# Autodesk Inventor assembly: Plate Assembly
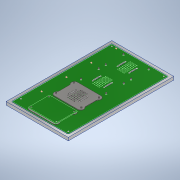
[picture p0: Inventor's stored thumbnail of the model, 180x180]
Saved by Autodesk Inventor 2022 (Build 260153000, 153)
## iProperties
Created: 2021-07-29
Part Number: Plate Assembly
Document SubType Name: Assembly
Designer: Caleb
Author: Caleb
## Documents named in this file (7)
- C:\Users\Caleb\Desktop\nebraska-silicon-lab\Hardware\ETL\Module Assembly\Tamale Assembly Plate V2\Plate Assembly.iam
- C:\Users\Caleb\Desktop\nebraska-silicon-lab\Hardware\ETL\Module Assembly\Tamale Assembly Plate V2\Tamale Assembly Plate.ipt
- C:\Users\Caleb\Desktop\nebraska-silicon-lab\Hardware\ETL\Module Assembly\Tamale Assembly Plate V2\91585A353_18-8 STAINLESS STEEL DOWEL PIN.ipt
- C:\Users\Caleb\Desktop\nebraska-silicon-lab\Hardware\ETL\Module Assembly\Tamale Assembly Plate V2\90910A443_BUTTON HEAD TORX SCREWS.ipt
- C:\Users\Caleb\Desktop\nebraska-silicon-lab\Hardware\ETL\Module Assembly\Tamale Assembly Plate V2\spacer.ipt
- C:\Users\Caleb\Desktop\nebraska-silicon-lab\Hardware\ETL\Module Assembly\Module PCB Mockup\etl_module_pcb_mockup_v1.iam
- C:\Users\Caleb\Desktop\nebraska-silicon-lab\Hardware\ETL\Module Assembly\Tamale Assembly Plate V2\etl_assembly_plate_pcb_v1.1\etl_assembly_plate_pcb_v1.iam
## Components (41 placed, 6 different names)
1. Tamale Assembly Plate:1 — Insert:1, Insert:2, Insert:3, Insert:4, Insert:5, Insert:6, Insert:7, Insert:8, Insert:9, Insert:10, Insert:11, Insert:12, Insert:13, Insert:14, Insert:15, Insert:16, Mate:5, Insert:17, Insert:18
2. 91585A353_18-8 STAINLESS STEEL DOWEL PIN:1 — Insert:2
3. 91585A353_18-8 STAINLESS STEEL DOWEL PIN:2 — Insert:3
4. 91585A353_18-8 STAINLESS STEEL DOWEL PIN:3 — Insert:4
5. 91585A353_18-8 STAINLESS STEEL DOWEL PIN:4 — Insert:1
6. 91585A353_18-8 STAINLESS STEEL DOWEL PIN:5 — Insert:8
7. 91585A353_18-8 STAINLESS STEEL DOWEL PIN:6 — Insert:7
8. 91585A353_18-8 STAINLESS STEEL DOWEL PIN:7 — Insert:6
9. 91585A353_18-8 STAINLESS STEEL DOWEL PIN:8 — Insert:5
10. 91585A353_18-8 STAINLESS STEEL DOWEL PIN:9 — Insert:9
11. 91585A353_18-8 STAINLESS STEEL DOWEL PIN:11 — Insert:10
12. 91585A353_18-8 STAINLESS STEEL DOWEL PIN:12 — Insert:16
13. 91585A353_18-8 STAINLESS STEEL DOWEL PIN:13 — Insert:15
14. 91585A353_18-8 STAINLESS STEEL DOWEL PIN:14 — Insert:13
15. 91585A353_18-8 STAINLESS STEEL DOWEL PIN:15 — Insert:12
16. 91585A353_18-8 STAINLESS STEEL DOWEL PIN:16 — Insert:11
17. 91585A353_18-8 STAINLESS STEEL DOWEL PIN:17 — Insert:14
18. spacer:1 — Mate:4
19. 90910A443_BUTTON HEAD TORX SCREWS:1
20. 90910A443_BUTTON HEAD TORX SCREWS:2
21. 90910A443_BUTTON HEAD TORX SCREWS:3
22. 90910A443_BUTTON HEAD TORX SCREWS:4
23. 90910A443_BUTTON HEAD TORX SCREWS:5
24. 90910A443_BUTTON HEAD TORX SCREWS:6
25. 90910A443_BUTTON HEAD TORX SCREWS:7
26. 90910A443_BUTTON HEAD TORX SCREWS:8
27. 90910A443_BUTTON HEAD TORX SCREWS:9
28. 90910A443_BUTTON HEAD TORX SCREWS:10
29. 90910A443_BUTTON HEAD TORX SCREWS:11
30. 90910A443_BUTTON HEAD TORX SCREWS:12
31. 90910A443_BUTTON HEAD TORX SCREWS:13
32. 90910A443_BUTTON HEAD TORX SCREWS:14
33. 90910A443_BUTTON HEAD TORX SCREWS:15
34. 90910A443_BUTTON HEAD TORX SCREWS:16
35. 90910A443_BUTTON HEAD TORX SCREWS:17
36. 90910A443_BUTTON HEAD TORX SCREWS:18
37. 90910A443_BUTTON HEAD TORX SCREWS:19
38. 90910A443_BUTTON HEAD TORX SCREWS:20
39. spacer:4
40. etl_module_pcb_mockup_v1:1 [sub-assembly] — Mate:4
41. etl_assembly_plate_pcb_v1:1 [sub-assembly] — Mate:5, Insert:17, Insert:18
## Relationships (20: Insert 18, Mate 2)
- Insert:1: Tamale Assembly Plate:1 ↔ 91585A353_18-8 STAINLESS STEEL DOWEL PIN:4
- Insert:2: Tamale Assembly Plate:1 ↔ 91585A353_18-8 STAINLESS STEEL DOWEL PIN:1
- Insert:3: Tamale Assembly Plate:1 ↔ 91585A353_18-8 STAINLESS STEEL DOWEL PIN:2
- Insert:4: Tamale Assembly Plate:1 ↔ 91585A353_18-8 STAINLESS STEEL DOWEL PIN:3
- Insert:5: Tamale Assembly Plate:1 ↔ 91585A353_18-8 STAINLESS STEEL DOWEL PIN:8
- Insert:6: Tamale Assembly Plate:1 ↔ 91585A353_18-8 STAINLESS STEEL DOWEL PIN:7
- Insert:7: Tamale Assembly Plate:1 ↔ 91585A353_18-8 STAINLESS STEEL DOWEL PIN:6
- Insert:8: Tamale Assembly Plate:1 ↔ 91585A353_18-8 STAINLESS STEEL DOWEL PIN:5
- Insert:9: Tamale Assembly Plate:1 ↔ 91585A353_18-8 STAINLESS STEEL DOWEL PIN:9
- Insert:10: Tamale Assembly Plate:1 ↔ 91585A353_18-8 STAINLESS STEEL DOWEL PIN:11
- Insert:11: Tamale Assembly Plate:1 ↔ 91585A353_18-8 STAINLESS STEEL DOWEL PIN:16
- Insert:12: Tamale Assembly Plate:1 ↔ 91585A353_18-8 STAINLESS STEEL DOWEL PIN:15
- Insert:13: Tamale Assembly Plate:1 ↔ 91585A353_18-8 STAINLESS STEEL DOWEL PIN:14
- Insert:14: Tamale Assembly Plate:1 ↔ 91585A353_18-8 STAINLESS STEEL DOWEL PIN:17
- Insert:15: Tamale Assembly Plate:1 ↔ 91585A353_18-8 STAINLESS STEEL DOWEL PIN:13
- Insert:16: Tamale Assembly Plate:1 ↔ 91585A353_18-8 STAINLESS STEEL DOWEL PIN:12
- Mate:4 (0.1 mm): spacer:1 ↔ etl_module_pcb_mockup_v1:1
- Mate:5: Tamale Assembly Plate:1 ↔ etl_assembly_plate_pcb_v1:1
- Insert:17: Tamale Assembly Plate:1 ↔ etl_assembly_plate_pcb_v1:1
- Insert:18: Tamale Assembly Plate:1 ↔ etl_assembly_plate_pcb_v1:1
